# Autodesk Inventor assembly: Threadded Stepper
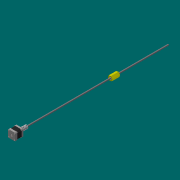
[picture p0: Inventor's stored thumbnail of the model, 180x180]
Saved by Autodesk Inventor 2016 (Build 200138000, 138)
## iProperties
Created: 2015-06-02
Part Number: Threadded Stepper
Document SubType Name: Assembly
Designer: Sawaiz Syed
Author: Sawaiz Syed
## Documents named in this file (5)
- C:\Users\Sawaiz\Documents\data\projects\cncBlackBox\xAxis\movementThreaddedAssembly.iam
- C:\Users\Sawaiz\Documents\data\projects\cncBlackBox\nema17Stepper\nema17.iam
- C:\Users\Sawaiz\Documents\data\projects\cncBlackBox\hardware\flexibleCoupling.ipt
- C:\Users\Sawaiz\Documents\data\projects\cncBlackBox\xAxis\xThreadedRod.ipt
- C:\Users\Sawaiz\Documents\data\projects\cncBlackBox\xAxis\antiBacklashNut.iam
## Components (4 placed, 4 different names)
1. nema17:1 [sub-assembly] — Mate:1, Flush:9
2. flexibleCoupling:1 — Mate:1, Flush:9, Mate:2, Mate:3
3. xThreadedRod:1 — Mate:2, Mate:3, Mate:4, Mate:5
4. antiBacklashNut:1 [sub-assembly] — Mate:4, Mate:5
## Relationships (6: Mate 5, Flush 1)
- Mate:1: nema17:1 ↔ flexibleCoupling:1
- Flush:9: nema17:1 ↔ flexibleCoupling:1
- Mate:2: flexibleCoupling:1 ↔ xThreadedRod:1
- Mate:3: flexibleCoupling:1 ↔ xThreadedRod:1
- Mate:4: xThreadedRod:1 ↔ antiBacklashNut:1
- Mate:5: xThreadedRod:1 ↔ antiBacklashNut:1
